# Autodesk Inventor assembly: gear20
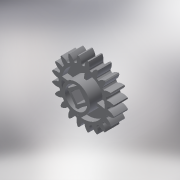
[picture p0: Inventor's stored thumbnail of the model, 180x180]
Saved by Autodesk Inventor 2019.3 (Build 233278000, 278)
## iProperties
Created: 2019-01-25
Part Number: gear20
Document SubType Name: Assembly
Designer: Varga Daniel
Author: Varga Daniel
## Documents named in this file (3)
- C:\!_Dani\!_cloud\OneDrive\!_munka\Revolution\RevvyDemoKit\Structural parts\Gears\G20.iam
- C:\!_Dani\!_cloud\OneDrive\!_munka\Revolution\RevvyDemoKit\Structural parts\Gears\gear20_tooth.ipt
- C:\!_Dani\!_cloud\OneDrive\!_munka\Revolution\RevvyDemoKit\Structural parts\Gears\gear_central_part_10.ipt
## Components (2 placed, 2 different names)
1. gear20_tooth:1 — Mate:1, Mate:2, Angle:1
2. gear_central_part_10:1 — Mate:1, Mate:2, Angle:1
## Relationships (3: Mate 2, Angle 1)
- Mate:1: gear20_tooth:1 ↔ gear_central_part_10:1
- Mate:2: gear20_tooth:1 ↔ gear_central_part_10:1
- Angle:1 (0 deg): gear20_tooth:1 ↔ gear_central_part_10:1
